# Autodesk Inventor assembly: assembly
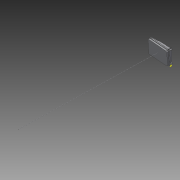
[picture p0: Inventor's stored thumbnail of the model, 180x180]
Saved by Autodesk Inventor 2015 SP1 (Build 190203100, 203)
## iProperties
Created: 2016-08-02
Part Number: assembly
Document SubType Name: Assembly
Designer: polidorop
Author: polidorop
## Documents named in this file (9)
- U:\git\idf\sleep_assay\hardware\inventor\assembly.iam
- U:\git\idf\sleep_assay\hardware\inventor\bottom_plate.ipt
- U:\git\idf\sleep_assay\hardware\inventor\top_plate.ipt
- U:\git\idf\sleep_assay\hardware\inventor\mount_plate.ipt
- U:\git\idf\sleep_assay\hardware\inventor\well_plate.ipt
- U:\git\idf\sleep_assay\hardware\inventor\angle_plate_long_tall.ipt
- U:\git\idf\sleep_assay\hardware\inventor\angle_plate_long_short.ipt
- U:\git\idf\sleep_assay\hardware\inventor\angle_plate_short_short.ipt
- U:\git\idf\sleep_assay\hardware\inventor\angle_plate_short_tall.ipt
## Components (11 placed, 8 different names)
1. bottom_plate:1 — Flush:1, Flush:2, Flush:3
2. top_plate:1 — Flush:4, Flush:5, Flush:6, Mate:1, Flush:7, Mate:2, Mate:3, Mate:4, Mate:5, Mate:6, Flush:8, Mate:7, Mate:8, Mate:9, Mate:10
3. mount_plate:1 — Mate:1, Flush:7, Mate:2, Mate:14, Mate:15, Mate:16, Mate:17, Mate:18, Mate:19, Mate:20, Mate:21, Mate:22, Mate:23, Mate:24, Flush:9, Mate:25, Mate:26, Flush:10
4. mount_plate:2 — Mate:3, Mate:4, Mate:5
5. mount_plate:3 — Mate:6, Flush:8, Mate:7
6. mount_plate:4 — Mate:8, Mate:9, Mate:10
7. well_plate:1 — Mate:13, Mate:14, Mate:15, Mate:16
8. angle_plate_long_tall:1 — Mate:17, Mate:18, Mate:19
9. angle_plate_long_short:1 — Mate:20, Mate:21, Mate:22
10. angle_plate_short_short:1 — Mate:23, Mate:24, Flush:9
11. angle_plate_short_tall:1 — Mate:25, Mate:26, Flush:10
## Relationships (34: Mate 24, Flush 10)
- Flush:1: bottom_plate:1
- Flush:2: bottom_plate:1
- Flush:3: bottom_plate:1
- Flush:4: top_plate:1
- Flush:5: top_plate:1
- Flush:6 (40 mm): top_plate:1
- Mate:1: top_plate:1 ↔ mount_plate:1
- Flush:7 (10 mm): top_plate:1 ↔ mount_plate:1
- Mate:2: top_plate:1 ↔ mount_plate:1
- Mate:3: top_plate:1 ↔ mount_plate:2
- Mate:4 (10 mm): top_plate:1 ↔ mount_plate:2
- Mate:5: top_plate:1 ↔ mount_plate:2
- Mate:6: top_plate:1 ↔ mount_plate:3
- Flush:8 (10 mm): top_plate:1 ↔ mount_plate:3
- Mate:7: top_plate:1 ↔ mount_plate:3
- Mate:8: top_plate:1 ↔ mount_plate:4
- Mate:9 (10 mm): top_plate:1 ↔ mount_plate:4
- Mate:10: top_plate:1 ↔ mount_plate:4
- Mate:13: well_plate:1
- Mate:14: mount_plate:1 ↔ well_plate:1
- Mate:15 (3 mm): mount_plate:1 ↔ well_plate:1
- Mate:16: mount_plate:1 ↔ well_plate:1
- Mate:17: mount_plate:1 ↔ angle_plate_long_tall:1
- Mate:18: mount_plate:1 ↔ angle_plate_long_tall:1
- Mate:19: mount_plate:1 ↔ angle_plate_long_tall:1
- Mate:20: mount_plate:1 ↔ angle_plate_long_short:1
- Mate:21: mount_plate:1 ↔ angle_plate_long_short:1
- Mate:22: mount_plate:1 ↔ angle_plate_long_short:1
- Mate:23: mount_plate:1 ↔ angle_plate_short_short:1
- Mate:24: mount_plate:1 ↔ angle_plate_short_short:1
- Flush:9: mount_plate:1 ↔ angle_plate_short_short:1
- Mate:25: mount_plate:1 ↔ angle_plate_short_tall:1
- Mate:26: mount_plate:1 ↔ angle_plate_short_tall:1
- Flush:10: mount_plate:1 ↔ angle_plate_short_tall:1
